# Autodesk Inventor assembly: OsnovanieWood
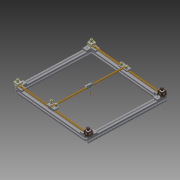
[picture p0: Inventor's stored thumbnail of the model, 180x180]
Saved by Autodesk Inventor 2015 (Build 190159000, 159)
## iProperties
Created: 2016-04-26
Part Number: OsnovanieWood
Document SubType Name: Assembly
Designer: Andreas
Author: Andreas
## Documents named in this file (16)
- C:\Users\criit\Desktop\проект\ласт_ворк_v1.5.3\Sborka.iam
- C:\Users\criit\Desktop\проект\ласт_ворк_v1.5.3\каркас\Balka.ipt
- C:\Users\criit\Desktop\проект\ласт_ворк_v1.5.3\каркас\Ugolok.ipt
- C:\Users\criit\Desktop\проект\ласт_ворк_v1.5.3\каркас\Relsa.ipt
- C:\Users\criit\Desktop\проект\ласт_ворк_v1.5.3\каретка+деталь к ней\Detal+Karetka.iam
- C:\Users\criit\Desktop\проект\ласт_ворк_v1.5.3\шпонька\Katushka.ipt
- C:\Users\criit\Desktop\проект\ласт_ворк_v1.5.3\мотор\Val.ipt
- C:\Users\criit\Desktop\проект\ласт_ворк_v1.5.3\мотор\Motor.ipt
- C:\Users\criit\Desktop\проект\ласт_ворк_v1.5.3\лазер\Laser.ipt
- C:\Users\criit\Desktop\проект\ласт_ворк_v1.5.3\лазер\ray.ipt
- C:\Users\criit\Desktop\проект\ласт_ворк_v1.5.3\шпонька\Podshipnik.ipt
- C:\Users\criit\Desktop\проект\ласт_ворк_v1.5.3\крепление\клешни\KleshnyaMotor.ipt
- C:\Users\criit\Desktop\проект\ласт_ворк_v1.5.3\крепление\KreplenieShpon.ipt
- C:\Users\criit\Desktop\проект\ласт_ворк_v1.5.3\шпонька\zaporkaShponki.ipt
- C:\Users\criit\Desktop\проект\ласт_ворк_v1.5.3\крепление\клешни\KleshnyaShpon.ipt
- C:\Users\criit\Desktop\проект\ласт_ворк_v1.5.3\новая каретка\NewKaretka.ipt
## Components (50 placed, 15 different names)
1. Balka:1 — Rigid:1, Rigid:2, Mate:1, Flush:1, Flush:2, Mate:62, Flush:36, Flush:37
2. Balka:2 — Rigid:1, Rigid:3
3. Balka:3 — Rigid:3, Flush:5, Flush:6, Mate:3, Mate:65, Flush:41, Flush:42
4. Balka:4 — Rigid:2
5. Ugolok:1 — Mate:1, Flush:1, Flush:2, Flush:9, Mate:34, Flush:34, Flush:35, Mate:53
6. Ugolok:2 — Mate:62, Flush:36, Flush:37, Mate:63, Flush:38, Flush:39, Mate:64, Mate:67, Flush:45
7. Ugolok:3 — Flush:5, Flush:6, Mate:3, Mate:5, Flush:10, Mate:87, Mate:90, Flush:52, Flush:53
8. Ugolok:4 — Mate:65, Flush:41, Flush:42, Mate:86, Mate:91, Flush:54, Flush:55
9. Relsa:1 — Mate:5, Flush:9, Flush:10, Mate:7, Mate:8
10. Relsa:2 — Mate:67, Flush:45, Mate:68, Mate:69, Mate:70
11. Detal+Karetka:1 [sub-assembly] — Mate:7, Mate:8, Flush:22, Flush:23, Mate:22, Flush:24, Mate:26, Mate:27, Mate:31, Mate:32, Mate:47, Mate:48, Mate:80, Tangent:17, Mate:81, Tangent:18
12. Relsa:3 — Flush:23, Mate:22, Flush:24, Mate:96, Mate:97
13. Katushka:2 — Mate:30, Rotational:9, Rotational:15, Mate:49
14. Katushka:3 — Tangent:7, Flush:46, Flush:47, Tangent:8
15. Katushka:5 — Mate:26, Mate:31, Rotational:7, Rotational:13, Mate:48
16. Katushka:6 — Mate:27, Mate:32, Rotational:6, Rotational:12, Mate:47
17. Katushka:11 — Cylindrical:19, Rotational:8, Rotational:14, Mate:50
18. Katushka:12 — Tangent:10, Mate:73, Mate:74, Tangent:11
19. Val:1 — Mate:43, Mate:44
20. Val:2 — Mate:41, Mate:42
21. Motor:1 — Mate:38, Mate:40, Mate:41, Mate:42, Mate:64
22. Motor:2 — Mate:43, Mate:44, Mate:51, Mate:52, Mate:53
23. Laser:1 — Rigid:18, Flush:56, Tangent:19
24. ray:1 — Rigid:18
25. Detal+Karetka:2 [sub-assembly] — Flush:22, Cylindrical:19, Mate:30, Mate:49, Mate:50, Mate:69, Mate:70, Mate:78, Tangent:15, Mate:79, Tangent:16
26. Podshipnik:1 — Mate:74, Tangent:11, Mate:75, Tangent:12
27. Podshipnik:2 — Rotational:14
28. Podshipnik:3 — Flush:47, Tangent:8, Mate:71
29. Podshipnik:4 — Rotational:13
30. Podshipnik:5 — Rotational:6
31. Podshipnik:7 — Rotational:12
32. Podshipnik:8 — Rotational:15
33. Podshipnik:9 — Tangent:10, Mate:73
34. Podshipnik:10 — Rotational:9
35. Podshipnik:11 — Tangent:7, Flush:46, Tangent:9
36. Podshipnik:12 — Rotational:7
37. Podshipnik:13 — Rotational:8
38. KleshnyaMotor:1 — Mate:38, Mate:40, Mate:63, Flush:38, Flush:39, Mate:68
39. KleshnyaMotor:2 — Mate:34, Flush:34, Flush:35, Mate:51, Mate:52
40. KreplenieShpon:1 — Tangent:9, Mate:71, Mate:76, Tangent:13, Mate:86, Mate:92, Mate:93
41. KreplenieShpon:2 — Mate:75, Tangent:12, Mate:77, Tangent:14, Mate:87, Mate:94, Mate:95
42. zaporkaShponki:1 — Mate:79, Tangent:16
43. zaporkaShponki:2 — Mate:76, Tangent:13
44. zaporkaShponki:3 — Mate:78, Tangent:15
45. zaporkaShponki:5 — Mate:77, Tangent:14
46. zaporkaShponki:6 — Mate:80, Tangent:17
47. zaporkaShponki:7 — Mate:81, Tangent:18
48. KleshnyaShpon:1 — Mate:91, Flush:54, Flush:55, Mate:92, Mate:93
49. KleshnyaShpon:2 — Mate:90, Flush:52, Flush:53, Mate:94, Mate:95
50. NewKaretka:1 — Mate:96, Mate:97, Flush:56, Tangent:19
## Relationships (104: Mate 53, Flush 25, Tangent 13, RevoluteJoint 8, WeldJoint 4, CylindricalJoint 1)
- Rigid:1 [WeldJoint]: Balka:1 ↔ Balka:2
- Rigid:2 [WeldJoint]: Balka:1 ↔ Balka:4
- Rigid:3 [WeldJoint]: Balka:2 ↔ Balka:3
- Mate:1: Balka:1 ↔ Ugolok:1
- Flush:1: Balka:1 ↔ Ugolok:1
- Flush:2: Balka:1 ↔ Ugolok:1
- Flush:5: Balka:3 ↔ Ugolok:3
- Flush:6: Balka:3 ↔ Ugolok:3
- Mate:3: Balka:3 ↔ Ugolok:3
- Mate:5: Ugolok:3 ↔ Relsa:1
- Flush:9 (-10 mm): Ugolok:1 ↔ Relsa:1
- Flush:10 (30 mm): Ugolok:3 ↔ Relsa:1
- Mate:7: Relsa:1 ↔ Detal+Karetka:1
- Mate:8: Relsa:1 ↔ Detal+Karetka:1
- Rigid:18 [WeldJoint]: Laser:1 ↔ ray:1
- Flush:22: Detal+Karetka:1 ↔ Detal+Karetka:2
- Flush:23 (-5 mm): Detal+Karetka:1 ↔ Relsa:3
- Mate:22: Detal+Karetka:1 ↔ Relsa:3
- Flush:24 (25 mm): Detal+Karetka:1 ↔ Relsa:3
- Mate:26: Detal+Karetka:1 ↔ Katushka:5
- Mate:27: Detal+Karetka:1 ↔ Katushka:6
- Cylindrical:19: Katushka:11 ↔ Detal+Karetka:2
- Mate:30: Katushka:2 ↔ Detal+Karetka:2
- Mate:31: Detal+Karetka:1 ↔ Katushka:5
- Mate:32: Detal+Karetka:1 ↔ Katushka:6
- Rotational:6 [RevoluteJoint]: Katushka:6 ↔ Podshipnik:5
- Rotational:7 [RevoluteJoint]: Katushka:5 ↔ Podshipnik:12
- Rotational:8 [RevoluteJoint]: Katushka:11 ↔ Podshipnik:13
- Rotational:9 [RevoluteJoint]: Katushka:2 ↔ Podshipnik:10
- Rotational:12 [RevoluteJoint]: Katushka:6 ↔ Podshipnik:7
- Rotational:13 [RevoluteJoint]: Katushka:5 ↔ Podshipnik:4
- Rotational:14 [RevoluteJoint]: Katushka:11 ↔ Podshipnik:2
- Rotational:15 [RevoluteJoint]: Katushka:2 ↔ Podshipnik:8
- Mate:34: Ugolok:1 ↔ KleshnyaMotor:2
- Mate:38: Motor:1 ↔ KleshnyaMotor:1
- Mate:40: Motor:1 ↔ KleshnyaMotor:1
- Mate:41: Val:2 ↔ Motor:1
- Mate:42: Val:2 ↔ Motor:1
- Mate:43: Val:1 ↔ Motor:2
- Mate:44: Val:1 ↔ Motor:2
- Mate:47: Detal+Karetka:1 ↔ Katushka:6
- Mate:48: Detal+Karetka:1 ↔ Katushka:5
- Mate:49: Katushka:2 ↔ Detal+Karetka:2
- Mate:50: Katushka:11 ↔ Detal+Karetka:2
- Flush:34: Ugolok:1 ↔ KleshnyaMotor:2
- Flush:35: Ugolok:1 ↔ KleshnyaMotor:2
- Mate:51: Motor:2 ↔ KleshnyaMotor:2
- Mate:52: Motor:2 ↔ KleshnyaMotor:2
- Mate:53: Ugolok:1 ↔ Motor:2
- Mate:62: Balka:1 ↔ Ugolok:2
- Flush:36: Balka:1 ↔ Ugolok:2
- Flush:37: Balka:1 ↔ Ugolok:2
- Mate:63: Ugolok:2 ↔ KleshnyaMotor:1
- Flush:38: Ugolok:2 ↔ KleshnyaMotor:1
- Flush:39: Ugolok:2 ↔ KleshnyaMotor:1
- Mate:64: Ugolok:2 ↔ Motor:1
- Mate:65: Balka:3 ↔ Ugolok:4
- Flush:41: Balka:3 ↔ Ugolok:4
- Flush:42: Balka:3 ↔ Ugolok:4
- Mate:67: Ugolok:2 ↔ Relsa:2
- Flush:45 (10 mm): Ugolok:2 ↔ Relsa:2
- Mate:68: Relsa:2 ↔ KleshnyaMotor:1
- Mate:69: Relsa:2 ↔ Detal+Karetka:2
- Mate:70: Relsa:2 ↔ Detal+Karetka:2
- Tangent:7: Katushka:3 ↔ Podshipnik:11
- Flush:46: Katushka:3 ↔ Podshipnik:11
- Flush:47: Katushka:3 ↔ Podshipnik:3
- Tangent:8: Katushka:3 ↔ Podshipnik:3
- Tangent:9: Podshipnik:11 ↔ KreplenieShpon:1
- Mate:71: Podshipnik:3 ↔ KreplenieShpon:1
- Tangent:10: Katushka:12 ↔ Podshipnik:9
- Mate:73: Katushka:12 ↔ Podshipnik:9
- Mate:74: Katushka:12 ↔ Podshipnik:1
- Tangent:11: Katushka:12 ↔ Podshipnik:1
- Mate:75: Podshipnik:1 ↔ KreplenieShpon:2
- Tangent:12: Podshipnik:1 ↔ KreplenieShpon:2
- Mate:76: KreplenieShpon:1 ↔ zaporkaShponki:2
- Tangent:13: KreplenieShpon:1 ↔ zaporkaShponki:2
- Mate:77: KreplenieShpon:2 ↔ zaporkaShponki:5
- Tangent:14: KreplenieShpon:2 ↔ zaporkaShponki:5
- Mate:78: Detal+Karetka:2 ↔ zaporkaShponki:3
- Tangent:15: Detal+Karetka:2 ↔ zaporkaShponki:3
- Mate:79: Detal+Karetka:2 ↔ zaporkaShponki:1
- Tangent:16: Detal+Karetka:2 ↔ zaporkaShponki:1
- Mate:80: Detal+Karetka:1 ↔ zaporkaShponki:6
- Tangent:17: Detal+Karetka:1 ↔ zaporkaShponki:6
- Mate:81: Detal+Karetka:1 ↔ zaporkaShponki:7
- Tangent:18: Detal+Karetka:1 ↔ zaporkaShponki:7
- Mate:86: Ugolok:4 ↔ KreplenieShpon:1
- Mate:87: Ugolok:3 ↔ KreplenieShpon:2
- Mate:90: Ugolok:3 ↔ KleshnyaShpon:2
- Flush:52: Ugolok:3 ↔ KleshnyaShpon:2
- Flush:53: Ugolok:3 ↔ KleshnyaShpon:2
- Mate:91: Ugolok:4 ↔ KleshnyaShpon:1
- Flush:54: Ugolok:4 ↔ KleshnyaShpon:1
- Flush:55: Ugolok:4 ↔ KleshnyaShpon:1
- Mate:92: KreplenieShpon:1 ↔ KleshnyaShpon:1
- Mate:93: KreplenieShpon:1 ↔ KleshnyaShpon:1
- Mate:94: KreplenieShpon:2 ↔ KleshnyaShpon:2
- Mate:95: KreplenieShpon:2 ↔ KleshnyaShpon:2
- Mate:96: Relsa:3 ↔ NewKaretka:1
- Mate:97: Relsa:3 ↔ NewKaretka:1
- Flush:56: Laser:1 ↔ NewKaretka:1
- Tangent:19: Laser:1 ↔ NewKaretka:1
